# Autodesk Inventor assembly: Anti-Spark
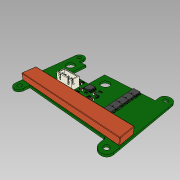
[picture p0: Inventor's stored thumbnail of the model, 180x180]
Saved by Autodesk Inventor 2018 (Build 220112000, 112)
## iProperties
Company: A Company
Created: 2019-09-10
Part Number: Anti-Spark
Description: KiCad electronic assembly
Document SubType Name: Assembly
Designer: vfv13
Authority: Unknown
Title: Anti-Spark.step
Author: An Author
Sending System: KiCad to STEP converter
Preprocessor: Open CASCADE STEP processor 6.9
## Documents named in this file (10)
- D:\Dokumente\Elektronik\Mountainboard\Anti-Spark\Anti-Spark\High-Side-NMOS-Antispark-Switch\Anti-Spark.iam
- D:\Dokumente\Elektronik\Mountainboard\Anti-Spark\Anti-Spark\High-Side-NMOS-Antispark-Switch\SOT1215.iam
- D:\Dokumente\Elektronik\Mountainboard\Anti-Spark\Anti-Spark\High-Side-NMOS-Antispark-Switch\TPS7A4101DGNR.iam
- D:\Dokumente\Elektronik\Mountainboard\Anti-Spark\Anti-Spark\High-Side-NMOS-Antispark-Switch\JST_XH_B4B-XH-A_1x04_P2.50mm_Vertical.iam
- D:\Dokumente\Elektronik\Mountainboard\Anti-Spark\Anti-Spark\High-Side-NMOS-Antispark-Switch\C_0805_2012Metric.iam
- D:\Dokumente\Elektronik\Mountainboard\Anti-Spark\Anti-Spark\High-Side-NMOS-Antispark-Switch\R_0805_2012Metric.iam
- D:\Dokumente\Elektronik\Mountainboard\Anti-Spark\Anti-Spark\High-Side-NMOS-Antispark-Switch\BQ76200PWR.iam
- D:\Dokumente\Elektronik\Mountainboard\Anti-Spark\Anti-Spark\High-Side-NMOS-Antispark-Switch\D_SOD-323.iam
- D:\Dokumente\Elektronik\Mountainboard\Anti-Spark\Anti-Spark\High-Side-NMOS-Antispark-Switch\COMPOUND_2.ipt
- D:\Dokumente\Part35.ipt
## Components (27 placed, 27 different names)
1. 2 [sub-assembly]
2. 3 [sub-assembly]
3. 4 [sub-assembly]
4. 5 [sub-assembly]
5. 6 [sub-assembly]
6. 7 [sub-assembly]
7. 8 [sub-assembly]
8. 9 [sub-assembly]
9. 10 [sub-assembly]
10. 11 [sub-assembly]
11. 13 [sub-assembly]
12. 15 [sub-assembly]
13. 17 [sub-assembly]
14. 19 [sub-assembly]
15. 20 [sub-assembly]
16. 21 [sub-assembly]
17. 23 [sub-assembly]
18. 24 [sub-assembly]
19. 25 [sub-assembly]
20. 26 [sub-assembly]
21. 28 [sub-assembly]
22. 29 [sub-assembly]
23. 30 [sub-assembly]
24. 31 [sub-assembly]
25. 32 [sub-assembly]
26. 33 — Flush:1, Flush:2
27. Part35:1 — Flush:1, Flush:2
## Relationships (2: Flush 2)
- Flush:1: 33 ↔ Part35:1
- Flush:2: 33 ↔ Part35:1
